# Autodesk Inventor assembly: trin
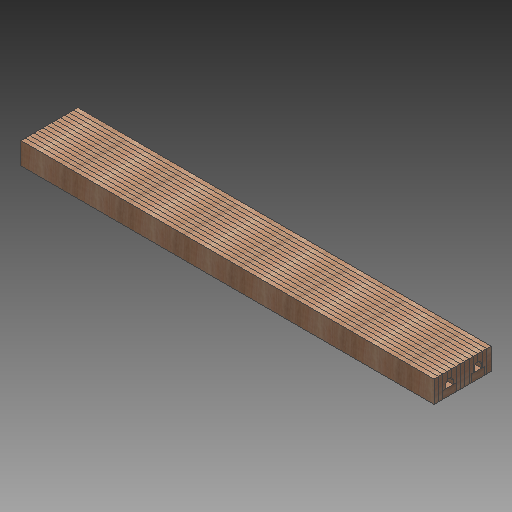
[picture p0: Inventor's stored thumbnail of the model, 512x512]
Saved by Autodesk Inventor 2018 (Build 220112000, 112)
## iProperties
Created: 2019-11-06
Part Number: trin
Document SubType Name: Assembly
Designer: loppen
Mass: 33872 g
Surface Area: 67826.8 cm^2
Volume: 46250.9 cm^3
Density: 0.732353 g/cm^3
Author: loppen
## Documents named in this file (4)
- Z:\trappe\trin\trin.iam
- Z:\trappe\trin\trinbrædt.ipt
- Z:\trappe\trin\trin-rør.ipt
- Z:\trappe\trin\liste.ipt
## Components (17 placed, 3 different names)
1. trinbrædt:1 — Mate:1, Flush:1, Flush:13, Flush:25, Flush:26, Flush:27
2. trinbrædt:2 — Mate:1, Mate:2, Flush:1, Flush:2, Flush:13, Flush:14
3. trinbrædt:3 — Mate:2, Mate:3, Flush:2, Flush:3, Flush:14, Flush:15, Mate:13
4. trinbrædt:4 — Mate:3, Mate:4, Flush:3, Flush:4, Flush:15, Flush:16
5. trinbrædt:5 — Mate:4, Mate:5, Flush:4, Flush:5, Flush:16, Flush:17, Mate:16, Mate:18
6. trinbrædt:6 — Mate:5, Mate:6, Flush:5, Flush:6, Flush:17, Flush:18
7. trinbrædt:7 — Mate:6, Mate:7, Flush:6, Flush:7, Flush:18, Flush:19
8. trinbrædt:8 — Mate:7, Mate:8, Flush:7, Flush:8, Flush:19, Flush:20
9. trinbrædt:9 — Mate:8, Mate:9, Flush:8, Flush:9, Flush:20, Flush:21
10. trinbrædt:10 — Mate:9, Mate:10, Flush:9, Flush:10, Flush:21, Flush:22, Mate:14
11. trinbrædt:11 — Mate:10, Mate:11, Flush:10, Flush:11, Flush:22, Flush:23
12. trinbrædt:12 — Mate:11, Flush:11, Mate:12, Flush:12, Flush:23, Flush:24, Mate:15, Mate:17
13. trinbrædt:13 — Mate:12, Flush:12, Flush:24
14. trin-rør:1 — Mate:13, Flush:25
15. trin-rør:2 — Mate:14, Flush:26
16. liste:1 — Mate:15, Mate:17, Flush:28
17. liste:2 — Mate:16, Mate:18, Flush:27, Flush:28
## Relationships (46: Flush 28, Mate 18)
- Mate:1: trinbrædt:1 ↔ trinbrædt:2
- Mate:2: trinbrædt:2 ↔ trinbrædt:3
- Mate:3: trinbrædt:3 ↔ trinbrædt:4
- Mate:4: trinbrædt:4 ↔ trinbrædt:5
- Mate:5: trinbrædt:5 ↔ trinbrædt:6
- Mate:6: trinbrædt:6 ↔ trinbrædt:7
- Mate:7: trinbrædt:7 ↔ trinbrædt:8
- Mate:8: trinbrædt:8 ↔ trinbrædt:9
- Mate:9: trinbrædt:9 ↔ trinbrædt:10
- Mate:10: trinbrædt:10 ↔ trinbrædt:11
- Mate:11: trinbrædt:11 ↔ trinbrædt:12
- Flush:1: trinbrædt:1 ↔ trinbrædt:2
- Flush:2: trinbrædt:2 ↔ trinbrædt:3
- Flush:3: trinbrædt:3 ↔ trinbrædt:4
- Flush:4: trinbrædt:4 ↔ trinbrædt:5
- Flush:5: trinbrædt:5 ↔ trinbrædt:6
- Flush:6: trinbrædt:6 ↔ trinbrædt:7
- Flush:7: trinbrædt:7 ↔ trinbrædt:8
- Flush:8: trinbrædt:8 ↔ trinbrædt:9
- Flush:9: trinbrædt:9 ↔ trinbrædt:10
- Flush:10: trinbrædt:10 ↔ trinbrædt:11
- Flush:11: trinbrædt:11 ↔ trinbrædt:12
- Mate:12: trinbrædt:12 ↔ trinbrædt:13
- Flush:12: trinbrædt:12 ↔ trinbrædt:13
- Flush:13: trinbrædt:1 ↔ trinbrædt:2
- Flush:14: trinbrædt:2 ↔ trinbrædt:3
- Flush:15: trinbrædt:3 ↔ trinbrædt:4
- Flush:16: trinbrædt:4 ↔ trinbrædt:5
- Flush:17: trinbrædt:5 ↔ trinbrædt:6
- Flush:18: trinbrædt:6 ↔ trinbrædt:7
- Flush:19: trinbrædt:7 ↔ trinbrædt:8
- Flush:20: trinbrædt:8 ↔ trinbrædt:9
- Flush:21: trinbrædt:9 ↔ trinbrædt:10
- Flush:22: trinbrædt:10 ↔ trinbrædt:11
- Flush:23: trinbrædt:11 ↔ trinbrædt:12
- Flush:24: trinbrædt:12 ↔ trinbrædt:13
- Mate:13: trinbrædt:3 ↔ trin-rør:1
- Mate:14: trinbrædt:10 ↔ trin-rør:2
- Flush:25: trinbrædt:1 ↔ trin-rør:1
- Flush:26: trinbrædt:1 ↔ trin-rør:2
- Mate:15: trinbrædt:12 ↔ liste:1
- Mate:16: trinbrædt:5 ↔ liste:2
- Mate:17: trinbrædt:12 ↔ liste:1
- Mate:18: trinbrædt:5 ↔ liste:2
- Flush:27: trinbrædt:1 ↔ liste:2
- Flush:28: liste:1 ↔ liste:2
